# Autodesk Inventor assembly: Ensemble_Boite_chassis
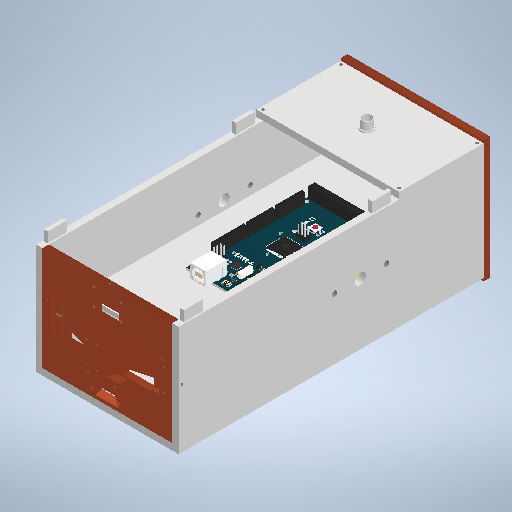
[picture p0: Inventor's stored thumbnail of the model, 512x512]
Saved by Autodesk Inventor 2026.2 (Build 302298010, 298A)
## iProperties
Created: 2026-03-16
Part Number: Ensemble_Boite_chassis
Document SubType Name: Assembly
Designer: genon
Author: genon
## Documents named in this file (11)
- C:\Users\genon\Documents\Henallux Passerelle\Projet de conception\Cassini T-X\Inventor\Ensemble_Boite_chassis.iam
- C:\Users\genon\Documents\Henallux Passerelle\Projet de conception\Cassini T-X\Inventor\chassis_bas.ipt
- C:\Users\genon\Documents\Henallux Passerelle\Projet de conception\Cassini T-X\Inventor\chassis_côté.ipt
- C:\Users\genon\Documents\Henallux Passerelle\Projet de conception\Cassini T-X\Inventor\chassis_face_arriere.ipt
- C:\Users\genon\Documents\Henallux Passerelle\Projet de conception\Cassini T-X\Inventor\chassis_haut.ipt
- C:\Users\genon\Documents\Henallux Passerelle\Projet de conception\Cassini T-X\Inventor\Composants\Arduino Mega 2560\Arduino Mega 2560\Arduino Mega 2560.ipt
- C:\Users\genon\Documents\Henallux Passerelle\Projet de conception\Cassini T-X\Inventor\Composants\Batterie.ipt
- C:\Users\genon\Documents\Henallux Passerelle\Projet de conception\Cassini T-X\Inventor\chassis arriere.ipt
- C:\Users\genon\Documents\Henallux Passerelle\Projet de conception\Cassini T-X\Inventor\Composants\Batterie 2.ipt
- C:\Users\genon\Documents\Henallux Passerelle\Projet de conception\Cassini T-X\Inventor\Support intérieur châssis.ipt
- C:\Users\genon\Documents\Henallux Passerelle\Projet de conception\Cassini T-X\Inventor\châssis haut avant.ipt
## Components (11 placed, 10 different names)
1. chassis_bas:1 — Placage:11, Placage:15, Placage:16, Placage:17, Placage:18, Placage:20, Placage:26, Placage:27, Placage:29, Placage:31, Placage:32, Placage:33, Placage:34
2. chassis_côté:1 — Placage:20, Placage:22, Placage:28, Placage:29, Placage:33, Placage:37, Placage:40
3. chassis_côté:2 — Placage:31, Placage:32, Placage:34, Placage:35, Placage:36, Placage:39
4. chassis_face_arriere:2 — Placage:26, Placage:27, Placage:28, Placage:41
5. chassis_haut:1 — Placage:22, Placage:35, Placage:38
6. Arduino Mega 2560:1 — Placage:19
7. Batterie:1 — Placage:11
8. chassis arriere:1 — Placage:36, Placage:37, Placage:38
9. Batterie 2:1 — Placage:15
10. Support intérieur châssis:1 — Placage:16, Placage:17, Placage:18, Placage:19
11. châssis haut avant:1 — Placage:39, Placage:40, Placage:41
## Relationships (23: Mate 23)
- Placage:11 [Mate]: chassis_bas:1 ↔ Batterie:1
- Placage:15 [Mate]: chassis_bas:1 ↔ Batterie 2:1
- Placage:16 [Mate]: chassis_bas:1 ↔ Support intérieur châssis:1
- Placage:17 [Mate]: chassis_bas:1 ↔ Support intérieur châssis:1
- Placage:18 [Mate]: chassis_bas:1 ↔ Support intérieur châssis:1
- Placage:19 [Mate]: Arduino Mega 2560:1 ↔ Support intérieur châssis:1
- Placage:20 [Mate]: chassis_bas:1 ↔ chassis_côté:1
- Placage:22 [Mate]: chassis_côté:1 ↔ chassis_haut:1
- Placage:26 [Mate]: chassis_bas:1 ↔ chassis_face_arriere:2
- Placage:27 [Mate]: chassis_bas:1 ↔ chassis_face_arriere:2
- Placage:28 [Mate]: chassis_côté:1 ↔ chassis_face_arriere:2
- Placage:29 [Mate]: chassis_bas:1 ↔ chassis_côté:1
- Placage:31 [Mate]: chassis_bas:1 ↔ chassis_côté:2
- Placage:32 [Mate]: chassis_bas:1 ↔ chassis_côté:2
- Placage:33 [Mate]: chassis_bas:1 ↔ chassis_côté:1
- Placage:34 [Mate]: chassis_bas:1 ↔ chassis_côté:2
- Placage:35 [Mate]: chassis_côté:2 ↔ chassis_haut:1
- Placage:36 [Mate]: chassis_côté:2 ↔ chassis arriere:1
- Placage:37 [Mate]: chassis_côté:1 ↔ chassis arriere:1
- Placage:38 [Mate] (0.05 mm): chassis_haut:1 ↔ chassis arriere:1
- Placage:39 [Mate]: chassis_côté:2 ↔ châssis haut avant:1
- Placage:40 [Mate]: chassis_côté:1 ↔ châssis haut avant:1
- Placage:41 [Mate]: chassis_face_arriere:2 ↔ châssis haut avant:1
